# Autodesk Inventor assembly: antenna_assembly_v3
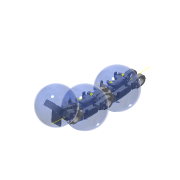
[picture p0: Inventor's stored thumbnail of the model, 180x180]
Saved by Autodesk Inventor 2017 (Build 210142000, 142)
## iProperties
Created: 2018-06-29
Part Number: antenna_assembly_v3
Document SubType Name: Assembly
Designer: Nic
Author: Nic
## Documents named in this file (6)
- C:\Users\Nic\Documents\Antenna\antenna_assembly_v3.iam
- C:\Users\Nic\Documents\Antenna\middle_segment_v3.ipt
- C:\Users\Nic\Documents\Antenna\end_segment_v3.ipt
- C:\Users\Nic\Documents\Antenna\sensor_pad_small.ipt
- C:\Users\Nic\Documents\Antenna\end_pad.ipt
- C:\Users\Nic\Documents\Antenna\prox_sensorIR.ipt
## Components (7 placed, 5 different names)
1. middle_segment_v3:1 — Insert:1, Insert:2, Mate:4, Flush:1, Flush:2, Mate:5
2. end_segment_v3:1 — Insert:1, Mate:2, Ball:1, Angle:1
3. middle_segment_v3:2 — Insert:2, Mate:6, Flush:3
4. sensor_pad_small:1 — Mate:6, Flush:3
5. sensor_pad_small:2 — Flush:2, Mate:5
6. end_pad:1 — Ball:1, Angle:1
7. prox_sensorIR:1 — Mate:4, Flush:1
## Relationships (11: Mate 4, Flush 3, Insert 2, BallJoint 1, Angle 1)
- Insert:1 (0.15 mm): middle_segment_v3:1 ↔ end_segment_v3:1
- Insert:2 (0.2 mm): middle_segment_v3:1 ↔ middle_segment_v3:2
- Mate:2: end_segment_v3:1
- Mate:4: middle_segment_v3:1 ↔ prox_sensorIR:1
- Flush:1 (-2 mm): middle_segment_v3:1 ↔ prox_sensorIR:1
- Ball:1: end_segment_v3:1 ↔ end_pad:1
- Angle:1 (180 deg): end_segment_v3:1 ↔ end_pad:1
- Flush:2 (-1 mm): middle_segment_v3:1 ↔ sensor_pad_small:2
- Mate:5: middle_segment_v3:1 ↔ sensor_pad_small:2
- Mate:6: middle_segment_v3:2 ↔ sensor_pad_small:1
- Flush:3 (-1 mm): middle_segment_v3:2 ↔ sensor_pad_small:1
